# Autodesk Inventor assembly: Gavrila r. P. Razvan stefan-T6
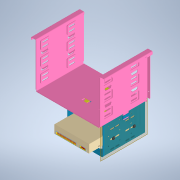
[picture p0: Inventor's stored thumbnail of the model, 180x180]
Saved by Autodesk Inventor 2022 (Build 260153000, 153)
## iProperties
Created: 2022-02-22
Part Number: Gavrila r. P. Razvan stefan-T6
Document SubType Name: Assembly
Designer: Anca Didu
Student_ACE: Gavrila r. P. Razvan stefan
Grupa_ACE: CR-1.2a
Tema_ACE: 6-Ansamblu suporti table
An_ACE: 2022
Author: Anca Didu
## Documents named in this file (6)
- C:\facultate\invertor projects\T6\Gavrila r. P. Razvan stefan-T6.iam
- C:\facultate\invertor projects\Gavrila r. P. Razvan stefan-T5.ipt
- C:\facultate\invertor projects\T6\CapacSuport.ipt
- C:\facultate\invertor projects\T6\SuportCD.ipt
- C:\facultate\invertor projects\T6\Hdd.ipt
- C:\Users\TheAl\Documents\Inventor\Content Center Files\R2022\en-US\ISO 7045  H\ISO 7045 - M4 x 5_ - 4.8 - H - ISO.ipt
## Components (8 placed, 5 different names)
1. Gavrila r. P. Razvan stefan-T5:1 — Flush:1, Flush:2, Flush:3, Flush:4, Mate:3, Mate:4, Angle:1, Mate:5, Mate:7, Mate:9, Mate:11
2. CapacSuport:1 — Flush:1, Flush:2, Flush:3, Mate:1, Mate:2
3. SuportCD:1 — Mate:1, Mate:2, Flush:4
4. Hdd:1 — Mate:3, Mate:4, Angle:1, Mate:6, Mate:8, Mate:10, Mate:12
5. ISO 7045 H M4 x 5 - 4.8 - H:1 — Mate:5, Mate:6
6. ISO 7045 H M4 x 5 - 4.8 - H:2 — Mate:9, Mate:10
7. ISO 7045 H M4 x 5 - 4.8 - H:3 — Mate:11, Mate:12
8. ISO 7045 H M4 x 5 - 4.8 - H:4 — Mate:7, Mate:8
## Relationships (17: Mate 12, Flush 4, Angle 1)
- Flush:1: Gavrila r. P. Razvan stefan-T5:1 ↔ CapacSuport:1
- Flush:2: Gavrila r. P. Razvan stefan-T5:1 ↔ CapacSuport:1
- Flush:3: Gavrila r. P. Razvan stefan-T5:1 ↔ CapacSuport:1
- Mate:1: CapacSuport:1 ↔ SuportCD:1
- Mate:2: CapacSuport:1 ↔ SuportCD:1
- Flush:4 (11 mm): Gavrila r. P. Razvan stefan-T5:1 ↔ SuportCD:1
- Mate:3 (-0.5 mm): Gavrila r. P. Razvan stefan-T5:1 ↔ Hdd:1
- Mate:4: Gavrila r. P. Razvan stefan-T5:1 ↔ Hdd:1
- Angle:1 (0 deg): Gavrila r. P. Razvan stefan-T5:1 ↔ Hdd:1
- Mate:5: Gavrila r. P. Razvan stefan-T5:1 ↔ ISO 7045 H M4 x 5 - 4.8 - H:1
- Mate:6: Hdd:1 ↔ ISO 7045 H M4 x 5 - 4.8 - H:1
- Mate:7: Gavrila r. P. Razvan stefan-T5:1 ↔ ISO 7045 H M4 x 5 - 4.8 - H:4
- Mate:8: Hdd:1 ↔ ISO 7045 H M4 x 5 - 4.8 - H:4
- Mate:9: Gavrila r. P. Razvan stefan-T5:1 ↔ ISO 7045 H M4 x 5 - 4.8 - H:2
- Mate:10: Hdd:1 ↔ ISO 7045 H M4 x 5 - 4.8 - H:2
- Mate:11: Gavrila r. P. Razvan stefan-T5:1 ↔ ISO 7045 H M4 x 5 - 4.8 - H:3
- Mate:12: Hdd:1 ↔ ISO 7045 H M4 x 5 - 4.8 - H:3
